# Autodesk Inventor assembly: ASY GBK bottom 0020
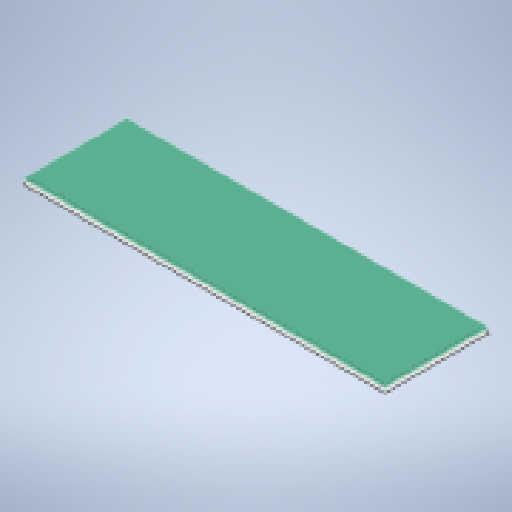
[picture p0: Inventor's stored thumbnail of the model, 512x512]
Saved by Autodesk Inventor 2026.2 (Build 302298000, 298)
## iProperties
Created: 2026-07-15
Part Number: ASY GBK bottom 0020
Document SubType Name: Assembly
Designer: admin
Author: admin
## Documents named in this file (4)
- C:\Users\user\Documents\Inventor\GBK-Gubkinskiy\ASY GBK bottom 0020.iam
- C:\Users\user\Documents\Inventor\GBK-Gubkinskiy\Пол\GBK bottom 0112.ipt
- C:\Users\user\Documents\Inventor\GBK-Gubkinskiy\Пол\GBK bottom 0135.ipt
- C:\Users\user\Documents\Inventor\GBK-Gubkinskiy\Пол\GBK bottom 0132.ipt
## Components (3 placed, 3 different names)
1. GBK bottom 0123:1
2. 0922_CPY1:1
3. 0923_CPY:1
## Relationships (4: Mate 3, WeldJoint 1)
- [WeldJoint]: 0922_CPY1:1 ↔ 0923_CPY:1
- [Mate]: GBK bottom 0123:1 ↔ 0923_CPY:1
- [Mate] (-30 mm): GBK bottom 0123:1 ↔ 0922_CPY1:1
- [Mate] (-30 mm): GBK bottom 0123:1 ↔ 0923_CPY:1
